# Autodesk Inventor assembly: maze_version2
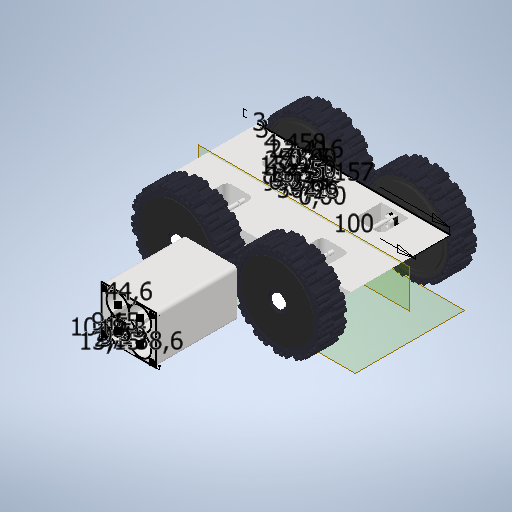
[picture p0: Inventor's stored thumbnail of the model, 512x512]
Saved by Autodesk Inventor 2025 (Build 290162000, 162)
## iProperties
Created: 2026-06-23
Part Number: maze_version2
Document SubType Name: Assembly
Designer: garin
Author: garin
## Documents named in this file (4)
- C:\Users\garin\Documents\Git\TheseusV2_Maze\Construction\Theseus_v2\Theseus_v2.iam
- C:\Users\garin\Documents\Git\TheseusV2_Maze\Construction\Theseus_v2\DDSM210.ipt
- C:\Users\garin\Documents\Git\TheseusV2_Maze\Construction\akkum_TSE\akkum.iam
- C:\Users\garin\Documents\Git\TheseusV2_Maze\Construction\akkum_TSE\low_part.ipt
## Components (6 placed, 3 different names)
1. low_part:1 — Заподлицо:1, Заподлицо:2, Заподлицо:3, Совмещение:1, Совмещение:2, Совмещение:3, Совмещение:7, Совмещение:8, Совмещение:9, Заподлицо:4, Совмещение:27, Совмещение:28, Совмещение:29, Совмещение:30, Совмещение:31, Совмещение:32
2. DDSM210:1 — Совмещение:27, Совмещение:28, Совмещение:29
3. DDSM210:2 — Совмещение:1, Совмещение:2, Совмещение:3
4. DDSM210:3 — Совмещение:30, Совмещение:31, Совмещение:32
5. DDSM210:4 — Совмещение:7, Совмещение:8, Совмещение:9
6. akkum:2 [sub-assembly]
## Relationships (16: Mate 12, Flush 4)
- Заподлицо:1 [Flush]: low_part:1
- Заподлицо:2 [Flush]: low_part:1
- Заподлицо:3 [Flush]: low_part:1
- Совмещение:1 [Mate]: low_part:1 ↔ DDSM210:2
- Совмещение:2 [Mate]: low_part:1 ↔ DDSM210:2
- Совмещение:3 [Mate]: low_part:1 ↔ DDSM210:2
- Совмещение:7 [Mate]: low_part:1 ↔ DDSM210:4
- Совмещение:8 [Mate]: low_part:1 ↔ DDSM210:4
- Совмещение:9 [Mate]: low_part:1 ↔ DDSM210:4
- Заподлицо:4 [Flush] (23 mm): low_part:1
- Совмещение:27 [Mate]: low_part:1 ↔ DDSM210:1
- Совмещение:28 [Mate]: low_part:1 ↔ DDSM210:1
- Совмещение:29 [Mate]: low_part:1 ↔ DDSM210:1
- Совмещение:30 [Mate]: low_part:1 ↔ DDSM210:3
- Совмещение:31 [Mate]: low_part:1 ↔ DDSM210:3
- Совмещение:32 [Mate]: low_part:1 ↔ DDSM210:3
